# Autodesk Inventor assembly: New_large_hinge_assembly
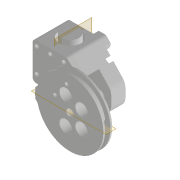
[picture p0: Inventor's stored thumbnail of the model, 180x180]
Saved by Autodesk Inventor 2022 (Build 260153000, 153)
## iProperties
Created: 2022-07-14
Part Number: New_large_hinge_assembly
Document SubType Name: Assembly
Designer: dell
Author: dell
## Documents named in this file (5)
- D:\xxxx\Uni\Part IV\MECHENG_700\Part_IV_project_CAD\Bird_skeleton_prototypes\Wing_drone_V1\Bird_wing_V2\New_large_hinge_assembly.iam
- D:\xxxx\Uni\Part IV\MECHENG_700\Part_IV_project_CAD\Bird_skeleton_prototypes\Wing_drone_V1\Bird_wing_V2\New_hinge.ipt
- D:\xxxx\Uni\Part IV\MECHENG_700\Part_IV_project_CAD\Bird_skeleton_prototypes\Wing_drone_V1\Bird_wing_V2\New_hinge_plate.ipt
- D:\xxxx\Uni\Part IV\MECHENG_700\Part_IV_project_CAD\Bird_skeleton_prototypes\Wing_drone_V1\Bird_wing_V2\New_coupling_pulley_p1.ipt
- D:\xxxx\Uni\Part IV\MECHENG_700\Part_IV_project_CAD\Bird_skeleton_prototypes\Wing_drone_V1\Bird_wing_V2\New_coupling_pulley_p2.ipt
## Components (6 placed, 4 different names)
1. New_hinge:1 — Mate:1, Mate:2, Mate:6, Mate:7, Mate:8
2. New_hinge:2 — Mate:1, Mate:2, Mate:3, Mate:4, Mate:5
3. New_hinge_plate:3 — Mate:3, Mate:4, Mate:5, Mate:12, Mate:13, Mate:14
4. New_hinge_plate:4 — Mate:6, Mate:7, Mate:8, Mate:15, Mate:16, Mate:17
5. New_coupling_pulley_p1:2 — Mate:12, Mate:13, Mate:14
6. New_coupling_pulley_p2:1 — Mate:15, Mate:16, Mate:17
## Relationships (14: Mate 14)
- Mate:1: New_hinge:1 ↔ New_hinge:2
- Mate:2: New_hinge:1 ↔ New_hinge:2
- Mate:3: New_hinge:2 ↔ New_hinge_plate:3
- Mate:4: New_hinge:2 ↔ New_hinge_plate:3
- Mate:5: New_hinge:2 ↔ New_hinge_plate:3
- Mate:6: New_hinge:1 ↔ New_hinge_plate:4
- Mate:7: New_hinge:1 ↔ New_hinge_plate:4
- Mate:8: New_hinge:1 ↔ New_hinge_plate:4
- Mate:12: New_hinge_plate:3 ↔ New_coupling_pulley_p1:2
- Mate:13: New_hinge_plate:3 ↔ New_coupling_pulley_p1:2
- Mate:14: New_hinge_plate:3 ↔ New_coupling_pulley_p1:2
- Mate:15: New_hinge_plate:4 ↔ New_coupling_pulley_p2:1
- Mate:16: New_hinge_plate:4 ↔ New_coupling_pulley_p2:1
- Mate:17: New_hinge_plate:4 ↔ New_coupling_pulley_p2:1
